# Autodesk Inventor assembly: A2017_T4_03
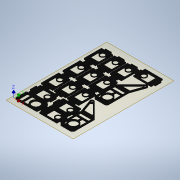
[picture p0: Inventor's stored thumbnail of the model, 180x180]
Saved by Autodesk Inventor 2022 (Build 260153000, 153)
## iProperties
Created: 2022-09-28
Part Number: A2017_T4_03
Document SubType Name: Assembly
Designer: Masato
Author: Masato
## Documents named in this file (6)
- C:\Users\ヨコオリク\Documents\CITBrains\SUSTAINA-OP\Cam\A2017_T4\A2017_T4_03.iam
- C:\Users\ヨコオリク\Documents\CITBrains\SUSTAINA-OP\Cam\DisposableBoard.ipt
- C:\Users\ヨコオリク\Documents\CITBrains\SUSTAINA-OP\UpperBody\Trunk\Trunk_neck_frame.ipt
- C:\Users\ヨコオリク\Documents\CITBrains\SUSTAINA-OP\UpperBody\Trunk\Trunk_shoulder_frame.ipt
- C:\Users\ヨコオリク\Documents\CITBrains\SUSTAINA-OP\UpperBody\Trunk\Trunk_shoulder_frame_MIR.ipt
- C:\Users\ヨコオリク\Documents\CITBrains\SUSTAINA-OP\UpperBody\Trunk\Trunk_servo_bottom_frame.ipt
## Components (17 placed, 5 different names)
1. DisposableBoard:1 — フラッシュ:1, フラッシュ:2, フラッシュ:3, フラッシュ:4, フラッシュ:11, フラッシュ:12, フラッシュ:13, フラッシュ:14, フラッシュ:15, フラッシュ:16, フラッシュ:17
2. Trunk_neck_frame:1 — メイト:3, メイト:7, フラッシュ:14, フラッシュ:15, メイト:20, メイト:29
3. Trunk_shoulder_frame:1 — メイト:2, フラッシュ:13, メイト:26
4. Trunk_shoulder_frame_MIR:1 — メイト:1, メイト:13, メイト:27, 正接:1
5. Trunk_servo_bottom_frame:1 — メイト:4, メイト:20, フラッシュ:16, メイト:24, メイト:26
6. Trunk_servo_bottom_frame:2 — メイト:5, メイト:24
7. Trunk_servo_bottom_frame:12 — メイト:17, メイト:18, フラッシュ:12, 正接:1
8. Trunk_servo_bottom_frame:13 — メイト:28, フラッシュ:17, メイト:29
9. Trunk_servo_bottom_frame:3 — メイト:14, フラッシュ:11
10. Trunk_servo_bottom_frame:4
11. Trunk_servo_bottom_frame:5 — メイト:27
12. Trunk_servo_bottom_frame:6
13. Trunk_servo_bottom_frame:7
14. Trunk_servo_bottom_frame:8
15. Trunk_servo_bottom_frame:9
16. Trunk_servo_bottom_frame:10
17. Trunk_servo_bottom_frame:11 — メイト:18
## Component patterns: (9 elements, first: Trunk_servo_bottom_frame:3)
## Relationships (28: Mate 16, Flush 11, Tangent 1)
- フラッシュ:1 [Flush]: DisposableBoard:1
- フラッシュ:2 [Flush]: DisposableBoard:1
- フラッシュ:3 [Flush]: DisposableBoard:1
- フラッシュ:4 [Flush]: DisposableBoard:1
- メイト:1 [Mate]: Trunk_shoulder_frame_MIR:1
- メイト:2 [Mate]: Trunk_shoulder_frame:1
- メイト:3 [Mate]: Trunk_neck_frame:1
- メイト:4 [Mate]: Trunk_servo_bottom_frame:1
- メイト:5 [Mate]: Trunk_servo_bottom_frame:2
- メイト:7 [Mate]: Trunk_neck_frame:1
- メイト:13 [Mate]: Trunk_shoulder_frame_MIR:1
- メイト:14 [Mate]: Trunk_servo_bottom_frame:3
- フラッシュ:11 [Flush] (2 mm): DisposableBoard:1 ↔ Trunk_servo_bottom_frame:3
- メイト:17 [Mate]: Trunk_servo_bottom_frame:12
- メイト:18 [Mate] (2.5 mm): Trunk_servo_bottom_frame:12 ↔ Trunk_servo_bottom_frame:11
- フラッシュ:12 [Flush] (2 mm): DisposableBoard:1 ↔ Trunk_servo_bottom_frame:12
- フラッシュ:13 [Flush] (2 mm): DisposableBoard:1 ↔ Trunk_shoulder_frame:1
- フラッシュ:14 [Flush] (2 mm): DisposableBoard:1 ↔ Trunk_neck_frame:1
- フラッシュ:15 [Flush] (2 mm): DisposableBoard:1 ↔ Trunk_neck_frame:1
- メイト:20 [Mate] (2.5 mm): Trunk_neck_frame:1 ↔ Trunk_servo_bottom_frame:1
- フラッシュ:16 [Flush] (2 mm): DisposableBoard:1 ↔ Trunk_servo_bottom_frame:1
- メイト:24 [Mate] (2.5 mm): Trunk_servo_bottom_frame:1 ↔ Trunk_servo_bottom_frame:2
- メイト:26 [Mate] (2.5 mm): Trunk_shoulder_frame:1 ↔ Trunk_servo_bottom_frame:1
- メイト:27 [Mate] (2.5 mm): Trunk_shoulder_frame_MIR:1 ↔ Trunk_servo_bottom_frame:5
- 正接:1 [Tangent] (3.5 mm): Trunk_shoulder_frame_MIR:1 ↔ Trunk_servo_bottom_frame:12
- メイト:28 [Mate]: Trunk_servo_bottom_frame:13
- フラッシュ:17 [Flush] (2 mm): DisposableBoard:1 ↔ Trunk_servo_bottom_frame:13
- メイト:29 [Mate] (2.5 mm): Trunk_neck_frame:1 ↔ Trunk_servo_bottom_frame:13
